# Autodesk Inventor assembly: stay22
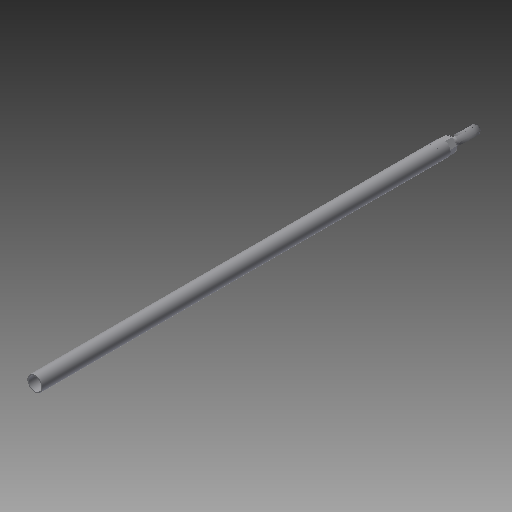
[picture p0: Inventor's stored thumbnail of the model, 512x512]
Saved by Autodesk Inventor 2018.3 (Build 223284000, 284)
## iProperties
Created: 2018-04-27
Part Number: stay22
Material: 一般
Document SubType Name: Assembly
Designer: ku_sk
Author: ku_sk
## Documents named in this file (3)
- D:\ku_sk\ドキュメント\Inventor\Aero\KS-15\Rr.wing\parts\stay\stay22.iam
- D:\ku_sk\ドキュメント\Inventor\Aero\KS-15\Rr.wing\parts\stay\pipe_16mm_420mm2.ipt
- D:\ku_sk\ドキュメント\Inventor\Aero\KS-15\Rr.wing\parts\stay\end\stay end2.iam
## Components (2 placed, 2 different names)
1. pipe_16mm_420mm2:1 — メイト:3, メイト:2, メイト:1, メイト:5, メイト:4
2. stay end2:1 [sub-assembly] — メイト:5, メイト:4
## Relationships (5: Mate 5)
- メイト:3 [Mate]: pipe_16mm_420mm2:1
- メイト:2 [Mate]: pipe_16mm_420mm2:1
- メイト:1 [Mate]: pipe_16mm_420mm2:1
- メイト:5 [Mate]: pipe_16mm_420mm2:1 ↔ stay end2:1
- メイト:4 [Mate]: pipe_16mm_420mm2:1 ↔ stay end2:1
